# Autodesk Inventor assembly: PWTR-0103
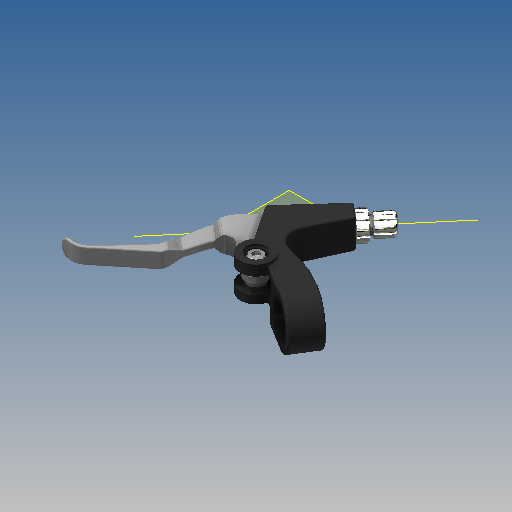
[picture p0: Inventor's stored thumbnail of the model, 512x512]
Saved by Autodesk Inventor 2021.1 (Build 251245000, 245)
## iProperties
Created: 2015-03-16
Part Number: PWTR-0103
Document SubType Name: Assembly
Designer: baris
Description: Control Lever
Author: baris
Revision Number: A
## Documents named in this file (8)
- C:\Vault Workspace\Design Data\Projects\PRJ0095\PWTR-CTO\PWTR-Supplier\PWTR-Controls\PWTR-0103.iam
- C:\Vault Workspace\Design Data\Projects\PRJ0095\PWTR-CTO\PWTR-Supplier\PWTR-Controls\PWTR-0110.ipt
- C:\Vault Workspace\Design Data\Projects\PRJ0095\PWTR-CTO\PWTR-Supplier\PWTR-Controls\PWTR-0109.ipt
- C:\Vault Workspace\Design Data\Projects\PRJ0095\PWTR-CTO\PWTR-Supplier\PWTR-Controls\PWTR-0106.ipt
- C:\Vault Workspace\Design Data\Projects\PRJ0095\PWTR-CTO\PWTR-Supplier\PWTR-Controls\PWTR-0104.ipt
- C:\Vault Workspace\Design Data\Projects\PRJ0095\PWTR-CTO\PWTR-Supplier\PWTR-Controls\PWTR-0105.ipt
- C:\Vault Workspace\Design Data\Projects\PRJ0095\PWTR-CTO\PWTR-Supplier\PWTR-Controls\PWTR-0107.ipt
- C:\Vault Workspace\Design Data\Projects\PRJ0095\PWTR-CTO\PWTR-Supplier\PWTR-Controls\PWTR-0108.ipt
## Components (7 placed, 7 different names)
1. PWTR-0110:1 — Mate:1, Mate:2, Cylindrical:1, Insert:1, Mate:4, Insert:2, Flush:1, Cylindrical:3
2. PWTR-0109:1 — Mate:2, Cylindrical:1
3. DIN 6912 M5 x 16:1 — Insert:1, Mate:3
4. Hex Jam Nut - Metric M5 x 0.8:1 — Mate:3, Mate:4
5. Broached Hexagon Socket Button Head Cap Screw - Metric M6 x 1 x 16:1 — Insert:2
6. PWTR-0107:1 — Flush:1, Cylindrical:3, Cylindrical:4
7. PWTR-0108:1 — Cylindrical:4
## Relationships (10: Mate 4, CylindricalJoint 3, Insert 2, Flush 1)
- Mate:1: PWTR-0110:1
- Mate:2 (2.5 mm): PWTR-0110:1 ↔ PWTR-0109:1
- Cylindrical:1: PWTR-0110:1 ↔ PWTR-0109:1
- Insert:1: PWTR-0110:1 ↔ DIN 6912 M5 x 16:1
- Mate:3: DIN 6912 M5 x 16:1 ↔ Hex Jam Nut - Metric M5 x 0.8:1
- Mate:4: PWTR-0110:1 ↔ Hex Jam Nut - Metric M5 x 0.8:1
- Insert:2: PWTR-0110:1 ↔ Broached Hexagon Socket Button Head Cap Screw - Metric M6 x 1 x 16:1
- Flush:1 (1.25 mm): PWTR-0110:1 ↔ PWTR-0107:1
- Cylindrical:3: PWTR-0110:1 ↔ PWTR-0107:1
- Cylindrical:4: PWTR-0107:1 ↔ PWTR-0108:1
